# Autodesk Inventor assembly: Chassis
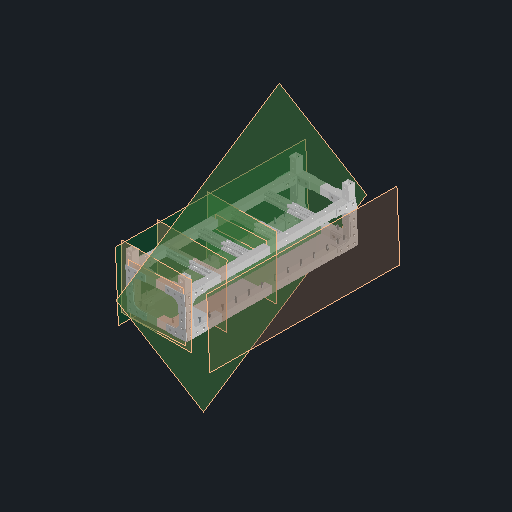
[picture p0: Inventor's stored thumbnail of the model, 512x512]
Saved by Autodesk Inventor 2024 (Build 280153000, 153)
## iProperties
Created: 2022-04-29
Part Number: Chassis
Document SubType Name: Assembly
Designer: Nebil Oumer
Mass: 8270.51 g
Surface Area: 16474 cm^2
Volume: 3063.15 cm^3
Density: 2.7 g/cm^3
Author: Nebil Oumer
## Documents named in this file (4)
- C:\Users\calvi\OneDrive\Robocup Rescue\Chassis\Frame\Centerpiece with DTconnector.iam
- Centerpiece.iam
- C:\Users\calvi\OneDrive\Robocup Rescue\Chassis\Frame\Centerpiece\Centerpiece_Frame.iam
- Centerpiece_Frame.iam
## Components (1 placed, 1 different names)
1. Centerpiece_Frame:1 [sub-assembly] — Flush:3, Flush:4, Symmetry:3, Symmetry:4
## Relationships (6: Flush 2, Symmetry 2, Mate 2)
- Flush:3: Centerpiece_Frame:1
- Flush:4: Centerpiece_Frame:1
- Symmetry:3: Centerpiece_Frame:1
- Symmetry:4: Centerpiece_Frame:1
- Mate:2
- Mate:3
